# Autodesk Inventor assembly: Final
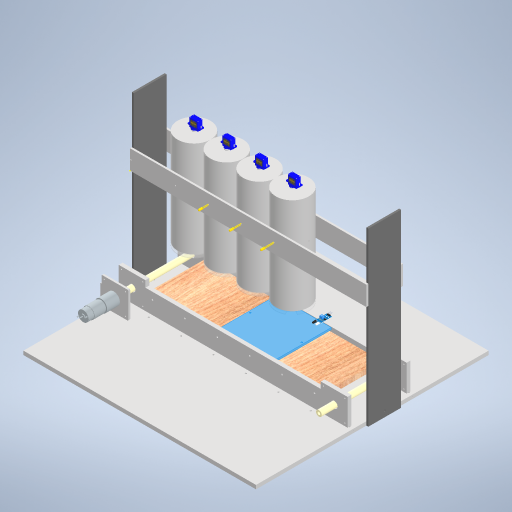
[picture p0: Inventor's stored thumbnail of the model, 512x512]
Saved by Autodesk Inventor 2023 (Build 270158000, 158)
## iProperties
Created: 2022-06-05
Part Number: Final
Document SubType Name: Assembly
Designer: prana_p9lsmih
Author: prana_p9lsmih
## Documents named in this file (18)
- E:\PRANAV\ENGINEERING EXPLORATION\VIRTUAL IMPLEMENTATION\3D Models\Final.iam
- E:\PRANAV\ENGINEERING EXPLORATION\VIRTUAL IMPLEMENTATION\3D Models\BASE.ipt
- E:\PRANAV\ENGINEERING EXPLORATION\VIRTUAL IMPLEMENTATION\3D Models\conveyor belt sideplank.ipt
- E:\PRANAV\ENGINEERING EXPLORATION\VIRTUAL IMPLEMENTATION\3D Models\Motor clamp p1.ipt
- E:\PRANAV\ENGINEERING EXPLORATION\VIRTUAL IMPLEMENTATION\3D Models\support.ipt
- E:\PRANAV\ENGINEERING EXPLORATION\VIRTUAL IMPLEMENTATION\3D Models\motor.ipt
- E:\PRANAV\ENGINEERING EXPLORATION\VIRTUAL IMPLEMENTATION\3D Models\shaft.ipt
- E:\PRANAV\ENGINEERING EXPLORATION\VIRTUAL IMPLEMENTATION\3D Models\belt support.ipt
- E:\PRANAV\ENGINEERING EXPLORATION\VIRTUAL IMPLEMENTATION\3D Models\support_seed_holder.ipt
- E:\PRANAV\ENGINEERING EXPLORATION\VIRTUAL IMPLEMENTATION\3D Models\side_support_holder.ipt
- E:\PRANAV\ENGINEERING EXPLORATION\VIRTUAL IMPLEMENTATION\3D Models\seed_holder.ipt
- E:\PRANAV\ENGINEERING EXPLORATION\VIRTUAL IMPLEMENTATION\3D Models\seed_disp_lid.ipt
- E:\PRANAV\ENGINEERING EXPLORATION\VIRTUAL IMPLEMENTATION\3D Models\extended_shaft.ipt
- E:\PRANAV\ENGINEERING EXPLORATION\VIRTUAL IMPLEMENTATION\3D Models\lid.ipt
- E:\PRANAV\ENGINEERING EXPLORATION\VIRTUAL IMPLEMENTATION\3D Models\parts\IRsensors.iam
- E:\PRANAV\ENGINEERING EXPLORATION\VIRTUAL IMPLEMENTATION\3D Models\parts\Ensamblaje.iam
- E:\PRANAV\ENGINEERING EXPLORATION\VIRTUAL IMPLEMENTATION\3D Models\pot_mover.ipt
- E:\PRANAV\ENGINEERING EXPLORATION\VIRTUAL IMPLEMENTATION\3D Models\parts\sg90-micro-servo-9g-tower-pro-1.snapshot.3\SG90 - Micro Servo 9g - Tower Pro.iam
## Components (47 placed, 17 different names)
1. BASE:1 — Mate:1, Mate:2, Mate:11, Mate:12, Mate:15, Mate:16, Mate:17, Mate:18, Mate:19, Flush:3, Mate:27, Mate:28, Mate:86, Mate:87, Flush:10
2. conveyor belt sideplank:1 — Mate:1, Mate:3, Mate:4, Mate:5, Mate:6, Mate:7, Mate:8, Mate:9, Mate:10, Mate:23, Mate:24, Mate:25, Mate:26
3. conveyor belt sideplank:2 — Mate:2, Mate:3, Mate:4, Mate:5, Mate:6, Mate:13, Mate:14, Flush:1, Flush:2, Mate:79, Mate:80, Mate:81, Mate:82, Mate:89
4. Motor clamp p1:1 — Mate:7, Mate:8, Mate:9, Mate:10, Mate:20, Mate:21
5. support:1 — Mate:18, Mate:19
6. support:2 — Mate:15, Mate:16, Mate:17
7. support:3 — Mate:11, Mate:12, Mate:13, Mate:14
8. motor:1 — Mate:20, Mate:21, Mate:22
9. shaft:1 — Mate:22, Flush:1
10. shaft:2 — Mate:23, Flush:2
11. belt support:1 — Mate:24, Mate:25, Mate:26
12. support_seed_holder:1 — Flush:3, Mate:27, Mate:28, Mate:29, Mate:30, Flush:4, Mate:31, Mate:32, Flush:5, Flush:6
13. side_support_holder:1 — Mate:29, Mate:30, Flush:4, Mate:33, Mate:34, Mate:35, Mate:36, Mate:83, Mate:84, Mate:85
14. side_support_holder:2 — Mate:31, Mate:32, Flush:5, Tangent:1, Tangent:2, Tangent:3, Tangent:4
15. seed_holder:1 — Mate:33, Tangent:1, Flush:6, Flush:7, Mate:37, Mate:38, Mate:39, Mate:49, Mate:70, Mate:74
16. seed_holder:2 — Mate:34, Tangent:2, Flush:7, Flush:8, Mate:40, Mate:41, Mate:48, Mate:50, Mate:71, Mate:75
17. seed_holder:3 — Mate:35, Tangent:3, Flush:8, Flush:9, Mate:42, Mate:43, Mate:47, Mate:53, Mate:72, Mate:76
18. seed_holder:4 — Mate:36, Tangent:4, Flush:9, Mate:44, Mate:45, Mate:46, Mate:52, Mate:73, Mate:88
19. seed_disp_lid:1 — Mate:37, Mate:38, Mate:39, Mate:57
20. seed_disp_lid:2 — Mate:40, Mate:41, Mate:48, Mate:61
21. seed_disp_lid:3 — Mate:42, Mate:43, Mate:47, Mate:65
22. seed_disp_lid:4 — Mate:44, Mate:45, Mate:46, Mate:69
23. extended_shaft:1 — Mate:49, Mate:54, Mate:55, Mate:56, Mate:93
24. extended_shaft:2 — Mate:50, Mate:58, Mate:59, Mate:60, Mate:92
25. extended_shaft:3 — Mate:53, Mate:62, Mate:63, Mate:64, Mate:91
26. extended_shaft:4 — Mate:52, Mate:66, Mate:67, Mate:68, Mate:90
27. seed_disp_lid:5 — Mate:54, Mate:55, Mate:56, Mate:57
28. seed_disp_lid:6 — Mate:58, Mate:59, Mate:60, Mate:61
29. seed_disp_lid:7 — Mate:62, Mate:63, Mate:64, Mate:65
30. seed_disp_lid:8 — Mate:66, Mate:67, Mate:68, Mate:69
31. lid:1 — Mate:70, Mate:74
32. lid:2 — Mate:71, Mate:75
33. lid:3 — Mate:72, Mate:76
34. lid:4 — Mate:73, Mate:88
35. IRsensors:1 [sub-assembly] — Mate:79
36. IRsensors:2 [sub-assembly] — Mate:80
37. IRsensors:3 [sub-assembly] — Mate:81
38. IRsensors:4 [sub-assembly] — Mate:82
39. Ensamblaje:2 [sub-assembly] — Mate:85
40. Ensamblaje:3 [sub-assembly] — Mate:84
41. Ensamblaje:4 [sub-assembly] — Mate:83
42. support_seed_holder:2 — Mate:86, Mate:87, Flush:10
43. pot_mover:1 — Mate:89
44. SG90 - Micro Servo 9g - Tower Pro:1 [sub-assembly] — Mate:93
45. SG90 - Micro Servo 9g - Tower Pro:2 [sub-assembly] — Mate:92
46. SG90 - Micro Servo 9g - Tower Pro:3 [sub-assembly] — Mate:91
47. SG90 - Micro Servo 9g - Tower Pro:4 [sub-assembly] — Mate:90
## Relationships (104: Mate 90, Flush 10, Tangent 4)
- Mate:1: BASE:1 ↔ conveyor belt sideplank:1
- Mate:2: BASE:1 ↔ conveyor belt sideplank:2
- Mate:3: conveyor belt sideplank:1 ↔ conveyor belt sideplank:2
- Mate:4: conveyor belt sideplank:1 ↔ conveyor belt sideplank:2
- Mate:5: conveyor belt sideplank:1 ↔ conveyor belt sideplank:2
- Mate:6 (145.029 mm): conveyor belt sideplank:1 ↔ conveyor belt sideplank:2
- Mate:7 (40 mm): conveyor belt sideplank:1 ↔ Motor clamp p1:1
- Mate:8: conveyor belt sideplank:1 ↔ Motor clamp p1:1
- Mate:9: conveyor belt sideplank:1 ↔ Motor clamp p1:1
- Mate:10: conveyor belt sideplank:1 ↔ Motor clamp p1:1
- Mate:11: BASE:1 ↔ support:3
- Mate:12: BASE:1 ↔ support:3
- Mate:13: conveyor belt sideplank:2 ↔ support:3
- Mate:14: conveyor belt sideplank:2 ↔ support:3
- Mate:15: BASE:1 ↔ support:2
- Mate:16: BASE:1 ↔ support:2
- Mate:17: BASE:1 ↔ support:2
- Mate:18: BASE:1 ↔ support:1
- Mate:19: BASE:1 ↔ support:1
- Mate:20: Motor clamp p1:1 ↔ motor:1
- Mate:21: Motor clamp p1:1 ↔ motor:1
- Mate:22: motor:1 ↔ shaft:1
- Flush:1: conveyor belt sideplank:2 ↔ shaft:1
- Mate:23: conveyor belt sideplank:1 ↔ shaft:2
- Flush:2: conveyor belt sideplank:2 ↔ shaft:2
- Mate:24: conveyor belt sideplank:1 ↔ belt support:1
- Mate:25: conveyor belt sideplank:1 ↔ belt support:1
- Mate:26: conveyor belt sideplank:1 ↔ belt support:1
- Flush:3: BASE:1 ↔ support_seed_holder:1
- Mate:27: BASE:1 ↔ support_seed_holder:1
- Mate:28: BASE:1 ↔ support_seed_holder:1
- Mate:29: support_seed_holder:1 ↔ side_support_holder:1
- Mate:30: support_seed_holder:1 ↔ side_support_holder:1
- Flush:4: support_seed_holder:1 ↔ side_support_holder:1
- Mate:31: support_seed_holder:1 ↔ side_support_holder:2
- Mate:32: support_seed_holder:1 ↔ side_support_holder:2
- Flush:5: support_seed_holder:1 ↔ side_support_holder:2
- Mate:33: side_support_holder:1 ↔ seed_holder:1
- Tangent:1: side_support_holder:2 ↔ seed_holder:1
- Flush:6: support_seed_holder:1 ↔ seed_holder:1
- Mate:34: side_support_holder:1 ↔ seed_holder:2
- Tangent:2: side_support_holder:2 ↔ seed_holder:2
- Flush:7: seed_holder:1 ↔ seed_holder:2
- Mate:35: side_support_holder:1 ↔ seed_holder:3
- Tangent:3: side_support_holder:2 ↔ seed_holder:3
- Flush:8: seed_holder:2 ↔ seed_holder:3
- Mate:36: side_support_holder:1 ↔ seed_holder:4
- Tangent:4: side_support_holder:2 ↔ seed_holder:4
- Flush:9: seed_holder:3 ↔ seed_holder:4
- Mate:37: seed_holder:1 ↔ seed_disp_lid:1
- Mate:38: seed_holder:1 ↔ seed_disp_lid:1
- Mate:39: seed_holder:1 ↔ seed_disp_lid:1
- Mate:40: seed_holder:2 ↔ seed_disp_lid:2
- Mate:41: seed_holder:2 ↔ seed_disp_lid:2
- Mate:42: seed_holder:3 ↔ seed_disp_lid:3
- Mate:43: seed_holder:3 ↔ seed_disp_lid:3
- Mate:44: seed_holder:4 ↔ seed_disp_lid:4
- Mate:45: seed_holder:4 ↔ seed_disp_lid:4
- Mate:46: seed_holder:4 ↔ seed_disp_lid:4
- Mate:47: seed_holder:3 ↔ seed_disp_lid:3
- Mate:48: seed_holder:2 ↔ seed_disp_lid:2
- Mate:49: seed_holder:1 ↔ extended_shaft:1
- Mate:50: seed_holder:2 ↔ extended_shaft:2
- Mate:52: seed_holder:4 ↔ extended_shaft:4
- Mate:53: seed_holder:3 ↔ extended_shaft:3
- Mate:54: extended_shaft:1 ↔ seed_disp_lid:5
- Mate:55: extended_shaft:1 ↔ seed_disp_lid:5
- Mate:56: extended_shaft:1 ↔ seed_disp_lid:5
- Mate:57 (5 mm): seed_disp_lid:1 ↔ seed_disp_lid:5
- Mate:58: extended_shaft:2 ↔ seed_disp_lid:6
- Mate:59: extended_shaft:2 ↔ seed_disp_lid:6
- Mate:60: extended_shaft:2 ↔ seed_disp_lid:6
- Mate:61 (5 mm): seed_disp_lid:2 ↔ seed_disp_lid:6
- Mate:62: extended_shaft:3 ↔ seed_disp_lid:7
- Mate:63: extended_shaft:3 ↔ seed_disp_lid:7
- Mate:64: extended_shaft:3 ↔ seed_disp_lid:7
- Mate:65 (5 mm): seed_disp_lid:3 ↔ seed_disp_lid:7
- Mate:66: extended_shaft:4 ↔ seed_disp_lid:8
- Mate:67: extended_shaft:4 ↔ seed_disp_lid:8
- Mate:68: extended_shaft:4 ↔ seed_disp_lid:8
- Mate:69 (5 mm): seed_disp_lid:4 ↔ seed_disp_lid:8
- Mate:70: seed_holder:1 ↔ lid:1
- Mate:71: seed_holder:2 ↔ lid:2
- Mate:72: seed_holder:3 ↔ lid:3
- Mate:73: seed_holder:4 ↔ lid:4
- Mate:74: seed_holder:1 ↔ lid:1
- Mate:75: seed_holder:2 ↔ lid:2
- Mate:76: seed_holder:3 ↔ lid:3
- Mate:79: conveyor belt sideplank:2 ↔ IRsensors:1
- Mate:80: conveyor belt sideplank:2 ↔ IRsensors:2
- Mate:81: conveyor belt sideplank:2 ↔ IRsensors:3
- Mate:82: conveyor belt sideplank:2 ↔ IRsensors:4
- Mate:83: side_support_holder:1 ↔ Ensamblaje:4
- Mate:84: side_support_holder:1 ↔ Ensamblaje:3
- Mate:85: side_support_holder:1 ↔ Ensamblaje:2
- Mate:86: BASE:1 ↔ support_seed_holder:2
- Mate:87: BASE:1 ↔ support_seed_holder:2
- Flush:10: BASE:1 ↔ support_seed_holder:2
- Mate:88: seed_holder:4 ↔ lid:4
- Mate:89: conveyor belt sideplank:2 ↔ pot_mover:1
- Mate:90: extended_shaft:4 ↔ SG90 - Micro Servo 9g - Tower Pro:4
- Mate:91: extended_shaft:3 ↔ SG90 - Micro Servo 9g - Tower Pro:3
- Mate:92: extended_shaft:2 ↔ SG90 - Micro Servo 9g - Tower Pro:2
- Mate:93: extended_shaft:1 ↔ SG90 - Micro Servo 9g - Tower Pro:1
